# Autodesk Inventor assembly: E006-Carter
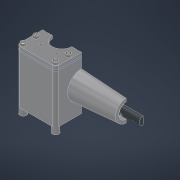
[picture p0: Inventor's stored thumbnail of the model, 180x180]
Saved by Autodesk Inventor 2021.3 (Build 253353000, 353)
## iProperties
Created: 2022-04-01
Part Number: E006-Carter
Document SubType Name: Assembly
Designer: remi
Author: remi
## Documents named in this file (18)
- C:\Users\remi\OneDrive\Documents\Cours\05-HEVS\S2fb\mechanic\CCo\project\Compressor\E006-Carter.iam
- C:\Users\remi\OneDrive\Documents\Cours\05-HEVS\S2fb\mechanic\CCo\project\Compressor\P016-Carter_corps.ipt
- C:\Users\remi\OneDrive\Documents\Cours\05-HEVS\S2fb\mechanic\CCo\project\Compressor\P015-Vilbrequin.ipt
- C:\Users\remi\OneDrive\Documents\Cours\05-HEVS\S2fb\mechanic\CCo\project\Compressor\P017-Carter_chapeau.ipt
- C:\Users\remi\OneDrive\Documents\Cours\05-HEVS\S2fb\mechanic\CCo\project\Compressor\P018-Joint_carter_chapeau.ipt
- C:\Users\remi\OneDrive\Documents\Cours\05-HEVS\S2fb\mechanic\CCo\project\Compressor\P020-Fixation_roulement_vilebrequin.ipt
- C:\Users\remi\OneDrive\Documents\Cours\05-HEVS\S2fb\mechanic\CCo\project\Compressor\R2021\en-US\AS 1420\AS 1420 - 1973 - M4 x 14.ipt
- C:\Users\remi\OneDrive\Documents\Cours\05-HEVS\S2fb\mechanic\CCo\project\Compressor\R2021\en-US\AS 1420\AS 1420 - 1973 - M4 x 8.ipt
- C:\Users\remi\OneDrive\Documents\Cours\05-HEVS\S2fb\mechanic\CCo\project\Compressor\P021-Bouchon_carter_vilbrequin.ipt
- C:\Users\remi\OneDrive\Documents\Cours\05-HEVS\S2fb\mechanic\CCo\project\Compressor\P022-Joint_carter_bouchon_vilbrequin.ipt
- C:\Users\remi\OneDrive\Documents\Cours\05-HEVS\S2fb\mechanic\CCo\project\Compressor\Roulements\AIS2021\SKF_W 61703-2RS1.iam
- C:\Users\remi\OneDrive\Documents\Cours\05-HEVS\S2fb\mechanic\CCo\project\Compressor\P024-Entretoise_roulements.ipt
- C:\Users\remi\OneDrive\Documents\Cours\05-HEVS\S2fb\mechanic\CCo\project\Compressor\E006-Carter\Design Accelerator\Key Connection2.iam
- C:\Users\remi\OneDrive\Documents\Cours\05-HEVS\S2fb\mechanic\CCo\project\Compressor\P025-Joint_carter_arbre.ipt
- C:\Users\remi\OneDrive\Documents\Cours\05-HEVS\S2fb\mechanic\CCo\project\Compressor\P026-Butée_carter_arbre.ipt
- C:\Users\remi\OneDrive\Documents\Cours\05-HEVS\S2fb\mechanic\CCo\project\Compressor\P023-Cage_arbre.ipt
- C:\Users\remi\OneDrive\Documents\Cours\05-HEVS\S2fb\mechanic\CCo\project\Compressor\R2021\en-US\AS 1420\AS 1420 - 1973 - M4 x 20.ipt
- C:\Users\remi\OneDrive\Documents\Cours\05-HEVS\S2fb\mechanic\CCo\project\Compressor\R2021\en-US\E 2076\_E 2076-10_.ipt
## Components (37 placed, 17 different names)
1. P016-Carter_corps:1 — Mate:6, Flush:1, Flush:2, Mate:9, Mate:10, Mate:11, Mate:16, Mate:22, Mate:23, Mate:24, Mate:25, Mate:28, Mate:31, Mate:35, Mate:37, Mate:38
2. P015-Vilbrequin:1 — Mate:7, Mate:8, Mate:14, Mate:15, Mate:18, Mate:20, Mate:31, Mate:34
3. P017-Carter_chapeau:1 — Mate:4, Mate:5, Flush:1, Flush:2, Insert:1, Insert:2, Insert:3, Insert:4, Insert:5, Insert:6, Insert:7, Insert:8
4. P018-Joint_carter_chapeau:1 — Mate:4, Mate:5, Mate:6
5. P020-Fixation_roulement_vilebrequin:1 — Mate:7, Mate:8, Insert:9
6. P021-Bouchon_carter_vilbrequin:1 — Mate:9, Insert:10, Insert:11, Insert:12, Insert:13, Insert:14, Insert:15
7. P022-Joint_carter_bouchon_vilbrequin:1 — Mate:10, Mate:11
8. P024-Entretoise_roulements:1 — Mate:20, Mate:21
9. Key Connection:1 [sub-assembly]
10. P025-Joint_carter_arbre:1 — Mate:22, Mate:25, Mate:32
11. P025-Joint_carter_arbre:2 — Mate:23, Mate:24, Mate:29, Mate:33
12. P026-Butée_carter_arbre:1 — Mate:28, Mate:29, Mate:30, Insert:16, Insert:17, Insert:18, Insert:19, Insert:20, Insert:21
13. P023-Cage_arbre:1 — Mate:34, Mate:35, Mate:36
14. E 2076 "14":1 — Mate:37, Mate:38
15. AS 1420 - Metric M4 x 20:1 — Insert:16
16. AS 1420 - Metric M4 x 20:2 — Insert:17
17. AS 1420 - Metric M4 x 20:3 — Insert:18
18. AS 1420 - Metric M4 x 20:4 — Insert:19
19. AS 1420 - Metric M4 x 20:5 — Insert:20
20. AS 1420 - Metric M4 x 20:6 — Insert:21
21. AS 1420 - Metric M4 x 8:2 — Insert:10
22. AS 1420 - Metric M4 x 8:3 — Insert:11
23. AS 1420 - Metric M4 x 8:4 — Insert:12
24. AS 1420 - Metric M4 x 8:5 — Insert:13
25. AS 1420 - Metric M4 x 8:6 — Insert:14
26. AS 1420 - Metric M4 x 8:7 — Insert:15
27. AS 1420 - Metric M4 x 14:1 — Insert:1
28. AS 1420 - Metric M4 x 14:2 — Insert:2
29. AS 1420 - Metric M4 x 14:3 — Insert:3
30. AS 1420 - Metric M4 x 14:4 — Insert:4
31. AS 1420 - Metric M4 x 14:5 — Insert:5
32. AS 1420 - Metric M4 x 14:6 — Insert:6
33. AS 1420 - Metric M4 x 14:7 — Insert:7
34. AS 1420 - Metric M4 x 14:8 — Insert:8
35. AS 1420 - Metric M4 x 8:1 — Insert:9
36. SKF_W 61703-2RS1:1 [sub-assembly] — Mate:14, Mate:15, Mate:16, Mate:21
37. SKF_W 61703-2RS1:2 [sub-assembly] — Mate:18
## Relationships (52: Mate 29, Insert 21, Flush 2)
- Mate:4: P017-Carter_chapeau:1 ↔ P018-Joint_carter_chapeau:1
- Mate:5: P017-Carter_chapeau:1 ↔ P018-Joint_carter_chapeau:1
- Mate:6: P016-Carter_corps:1 ↔ P018-Joint_carter_chapeau:1
- Flush:1: P016-Carter_corps:1 ↔ P017-Carter_chapeau:1
- Flush:2: P016-Carter_corps:1 ↔ P017-Carter_chapeau:1
- Mate:7: P015-Vilbrequin:1 ↔ P020-Fixation_roulement_vilebrequin:1
- Mate:8: P015-Vilbrequin:1 ↔ P020-Fixation_roulement_vilebrequin:1
- Insert:1: P017-Carter_chapeau:1 ↔ AS 1420 - Metric M4 x 14:1
- Insert:2: P017-Carter_chapeau:1 ↔ AS 1420 - Metric M4 x 14:2
- Insert:3: P017-Carter_chapeau:1 ↔ AS 1420 - Metric M4 x 14:3
- Insert:4: P017-Carter_chapeau:1 ↔ AS 1420 - Metric M4 x 14:4
- Insert:5: P017-Carter_chapeau:1 ↔ AS 1420 - Metric M4 x 14:5
- Insert:6: P017-Carter_chapeau:1 ↔ AS 1420 - Metric M4 x 14:6
- Insert:7: P017-Carter_chapeau:1 ↔ AS 1420 - Metric M4 x 14:7
- Insert:8: P017-Carter_chapeau:1 ↔ AS 1420 - Metric M4 x 14:8
- Insert:9: P020-Fixation_roulement_vilebrequin:1 ↔ AS 1420 - Metric M4 x 8:1
- Mate:9 (2 mm): P016-Carter_corps:1 ↔ P021-Bouchon_carter_vilbrequin:1
- Mate:10: P016-Carter_corps:1 ↔ P022-Joint_carter_bouchon_vilbrequin:1
- Mate:11: P016-Carter_corps:1 ↔ P022-Joint_carter_bouchon_vilbrequin:1
- Insert:10: P021-Bouchon_carter_vilbrequin:1 ↔ AS 1420 - Metric M4 x 8:2
- Insert:11: P021-Bouchon_carter_vilbrequin:1 ↔ AS 1420 - Metric M4 x 8:3
- Insert:12: P021-Bouchon_carter_vilbrequin:1 ↔ AS 1420 - Metric M4 x 8:4
- Insert:13: P021-Bouchon_carter_vilbrequin:1 ↔ AS 1420 - Metric M4 x 8:5
- Insert:14: P021-Bouchon_carter_vilbrequin:1 ↔ AS 1420 - Metric M4 x 8:6
- Insert:15: P021-Bouchon_carter_vilbrequin:1 ↔ AS 1420 - Metric M4 x 8:7
- Mate:14: P015-Vilbrequin:1 ↔ SKF_W 61703-2RS1:1
- Mate:15: P015-Vilbrequin:1 ↔ SKF_W 61703-2RS1:1
- Mate:16: P016-Carter_corps:1 ↔ SKF_W 61703-2RS1:1
- Mate:18: P015-Vilbrequin:1 ↔ SKF_W 61703-2RS1:2
- Mate:20: P015-Vilbrequin:1 ↔ P024-Entretoise_roulements:1
- Mate:21: P024-Entretoise_roulements:1 ↔ SKF_W 61703-2RS1:1
- Mate:22: P016-Carter_corps:1 ↔ P025-Joint_carter_arbre:1
- Mate:23: P016-Carter_corps:1 ↔ P025-Joint_carter_arbre:2
- Mate:24: P016-Carter_corps:1 ↔ P025-Joint_carter_arbre:2
- Mate:25: P016-Carter_corps:1 ↔ P025-Joint_carter_arbre:1
- Mate:28: P016-Carter_corps:1 ↔ P026-Butée_carter_arbre:1
- Mate:29: P025-Joint_carter_arbre:2 ↔ P026-Butée_carter_arbre:1
- Mate:30: P026-Butée_carter_arbre:1
- Mate:31: P016-Carter_corps:1 ↔ P015-Vilbrequin:1
- Mate:32: P025-Joint_carter_arbre:1
- Mate:33: P025-Joint_carter_arbre:2
- Mate:34: P015-Vilbrequin:1 ↔ P023-Cage_arbre:1
- Mate:35: P016-Carter_corps:1 ↔ P023-Cage_arbre:1
- Mate:36: P023-Cage_arbre:1
- Insert:16: P026-Butée_carter_arbre:1 ↔ AS 1420 - Metric M4 x 20:1
- Insert:17: P026-Butée_carter_arbre:1 ↔ AS 1420 - Metric M4 x 20:2
- Insert:18: P026-Butée_carter_arbre:1 ↔ AS 1420 - Metric M4 x 20:3
- Insert:19: P026-Butée_carter_arbre:1 ↔ AS 1420 - Metric M4 x 20:4
- Insert:20: P026-Butée_carter_arbre:1 ↔ AS 1420 - Metric M4 x 20:5
- Insert:21: P026-Butée_carter_arbre:1 ↔ AS 1420 - Metric M4 x 20:6
- Mate:37: P016-Carter_corps:1 ↔ E 2076 "14":1
- Mate:38: P016-Carter_corps:1 ↔ E 2076 "14":1
